# Autodesk Inventor assembly: 1stCutAtChainDrivenSystem
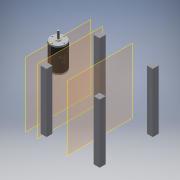
[picture p0: Inventor's stored thumbnail of the model, 180x180]
Saved by Autodesk Inventor 2016 SP1 (Build 200210100, 210)
## iProperties
Created: 2016-01-21
Part Number: 1stCutAtChainDrivenSystem
Document SubType Name: Assembly
Designer: steele
Author: steele
## Documents named in this file (3)
- C:\snobotics\CAD-Development\robSteele\SnoBotics2016\2ndCutAtPitchingMachineRobot\1stCutAtChainDrivenSystem.iam
- C:\snobotics\CAD-Development\robSteele\SnoBotics2016\2ndCutAtPitchingMachineRobot\VeryBasicFrame.ipt
- C:\snobotics\autodesk\2015\FRC_KOP_2015\Motors\MOT_CIM-Motor_217-2000.iam
## Components (2 placed, 2 different names)
1. VeryBasicFrame:1 — Flush:1, Flush:2
2. MOT_CIM-Motor_217-2000:1 [sub-assembly] — Flush:1, Mate:1, Flush:2
## Relationships (3: Flush 2, Mate 1)
- Flush:1: VeryBasicFrame:1 ↔ MOT_CIM-Motor_217-2000:1
- Mate:1: MOT_CIM-Motor_217-2000:1
- Flush:2: VeryBasicFrame:1 ↔ MOT_CIM-Motor_217-2000:1
